# Autodesk Inventor assembly: BG401_trajan20_21
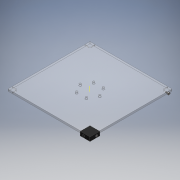
[picture p0: Inventor's stored thumbnail of the model, 180x180]
Saved by Autodesk Inventor 2022.2 (Build 262287000, 287)
## iProperties
Company: HTBLA Kaindorf
RuleStatus: InUse
Created: 2022-08-22
Part Number: BG401_trajan20_21
Project: Zeichenmaschine_v2
Material: Generisch
Description: papierplatte
Document SubType Name: Assembly
Designer: trajan20
AfterDocNew0: iProperties-Editor_aufrufen
Author: jan
Keywords: 2021
## Documents named in this file (5)
- C:\Users\jan\Documents\DrawMachine\DrawMachineConstruction\Projekt\Zeichenmaschine_v2\BG401_trajan20_21_Zeichenmaschine_v2_papierplatte.iam
- C:\Users\jan\Documents\DrawMachine\DrawMachineConstruction\Projekt\Zeichenmaschine_v2\BT403_trajan20_21_Zeichenmaschine_v2_papierplatte_plexi.ipt
- C:\Users\jan\Documents\DrawMachine\DrawMachineConstruction\Projekt\Zeichenmaschine_v2\BT406_trajan20_21_Zeichenmaschine_v2_Ecken.ipt
- C:\Users\jan\Documents\DrawMachine\DrawMachineConstruction\Projekt\Zeichenmaschine_v2\Normteile\de-DE\ISO 4762(2)\ISO 4762 - M3 x 5ISO.ipt
- C:\Users\jan\Documents\DrawMachine\DrawMachineConstruction\Projekt\Zeichenmaschine_v2\Normteile\de-DE\ISO 4762(2)\ISO 4762 - M3 x 8ISO.ipt
## Components (4 placed, 4 different names)
1. BT403_trajan20_21_Zeichenmaschine_v2_papierplatte_plexi:1 — Passend:1, Passend:2, Passend:3, Passend:5
2. BT406_trajan20_21_Zeichenmaschine_v2_Ecken:1 — Passend:1, Passend:2, Passend:4, Passend:6
3. ISO 4762 M3 x 8:1 — Passend:3, Passend:4
4. ISO 4762 M3 x 5:2 — Passend:5, Passend:6
## Relationships (6: Mate 6)
- Passend:1 [Mate]: BT403_trajan20_21_Zeichenmaschine_v2_papierplatte_plexi:1 ↔ BT406_trajan20_21_Zeichenmaschine_v2_Ecken:1
- Passend:2 [Mate]: BT403_trajan20_21_Zeichenmaschine_v2_papierplatte_plexi:1 ↔ BT406_trajan20_21_Zeichenmaschine_v2_Ecken:1
- Passend:3 [Mate]: BT403_trajan20_21_Zeichenmaschine_v2_papierplatte_plexi:1 ↔ ISO 4762 M3 x 8:1
- Passend:4 [Mate]: BT406_trajan20_21_Zeichenmaschine_v2_Ecken:1 ↔ ISO 4762 M3 x 8:1
- Passend:5 [Mate]: BT403_trajan20_21_Zeichenmaschine_v2_papierplatte_plexi:1 ↔ ISO 4762 M3 x 5:2
- Passend:6 [Mate]: BT406_trajan20_21_Zeichenmaschine_v2_Ecken:1 ↔ ISO 4762 M3 x 5:2
